# Autodesk Inventor assembly: Door Assembly
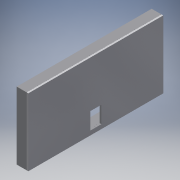
[picture p0: Inventor's stored thumbnail of the model, 180x180]
Saved by Autodesk Inventor 2017 (Build 210142000, 142)
## iProperties
Created: 2017-05-30
Part Number: Door Assembly
Document SubType Name: Assembly
Designer: cas7
Author: cas7
## Documents named in this file (4)
- C:\Users\Public\Documents\Autodesk\.desktop-connect\.docstore\guided-tutorial-plugin\INVNTOR\Compartment Modeling\Door Assembly.iam
- C:\Users\Public\Documents\Autodesk\.desktop-connect\.docstore\guided-tutorial-plugin\INVNTOR\Compartment Modeling\48in 2x4.ipt
- C:\Users\Public\Documents\Autodesk\.desktop-connect\.docstore\guided-tutorial-plugin\INVNTOR\2017\ENU\552100320579484105\TutorialModelPath\21in 2x4.ipt
- C:\Users\Public\Documents\Autodesk\.desktop-connect\.docstore\guided-tutorial-plugin\INVNTOR\Compartment Modeling\Door Gyp Board.ipt
## Components (7 placed, 2 different names)
1. 4ft 2x4:1
2. 4ft 2x4:2 — Mate:13
3. 4ft 2x4:3
4. 4ft 2x4:4
5. 4ft 2x4:5
6. 4ft 2x4:6 — Mate:12, Mate:14
7. Door Gyp Board:1 — Mate:12, Mate:13, Mate:14
## Relationships (14: Mate 14)
- [Mate]: 4ft 2x4:1 ↔ 4ft 2x4:2
- [Mate]: 4ft 2x4:1 ↔ 4ft 2x4:2
- [Mate]: 4ft 2x4:1 ↔ 4ft 2x4:2
- [Mate]: 4ft 2x4:1 ↔ 4ft 2x4:3
- [Mate]: 4ft 2x4:1 ↔ 4ft 2x4:3
- [Mate]: 4ft 2x4:1 ↔ 4ft 2x4:4
- [Mate]: 4ft 2x4:1 ↔ 4ft 2x4:5
- [Mate]: 4ft 2x4:2 ↔ 4ft 2x4:6
- [Mate]: 4ft 2x4:2 ↔ 4ft 2x4:6
- [Mate]: 4ft 2x4:5 ↔ 4ft 2x4:6
- [Mate]: 4ft 2x4:4 ↔ 4ft 2x4:6
- Mate:12: 4ft 2x4:6 ↔ Door Gyp Board:1
- Mate:13: 4ft 2x4:2 ↔ Door Gyp Board:1
- Mate:14: 4ft 2x4:6 ↔ Door Gyp Board:1
## Named parameters: d6_d8 = 0 mm, d7_d10 = 0 mm
